# Autodesk Inventor assembly: Battery holder assembly
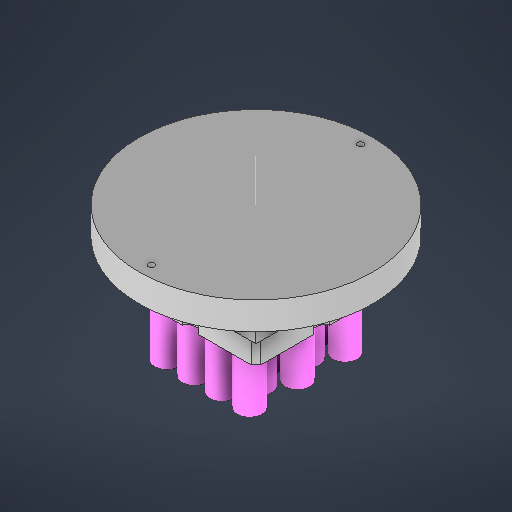
[picture p0: Inventor's stored thumbnail of the model, 512x512]
Saved by Autodesk Inventor 2025 (Build 290162000, 162)
## iProperties
Created: 2025-08-08
Part Number: Battery holder assembly
Document SubType Name: Assembly
Designer: mayhe
Author: mayhe
## Documents named in this file (4)
- C:\Users\mayhe\OneDrive\Documents\GitHub\In-situ-monitoring-of-powder-bed-fusion-additive-manufacturing\accessories\Battery Holder\Battery holder assembly.iam
- C:\Users\mayhe\OneDrive\Documents\GitHub\In-situ-monitoring-of-powder-bed-fusion-additive-manufacturing\accessories\threaded_build-plate\substrate plate With Lots of holes.ipt
- C:\Users\mayhe\OneDrive\Documents\GitHub\In-situ-monitoring-of-powder-bed-fusion-additive-manufacturing\accessories\Battery Holder\Battery Holder.ipt
- C:\Users\mayhe\OneDrive\Documents\GitHub\In-situ-monitoring-of-powder-bed-fusion-additive-manufacturing\accessories\Battery Holder\18650(PINK).ipt
## Components (20 placed, 3 different names)
1. substrate plate With Lots of holes:1 — Rotational:3, Mate:1
2. Battery Holder:1 — Rotational:2, Rotational:3, Mate:1, Rotational:4, Rotational:5, Rotational:6, Rotational:7, Rotational:8, Rotational:9, Rotational:10, Rotational:11, Rotational:12, Rigid:1, Rotational:13, Rigid:2, Rotational:14, Rotational:15, Rigid:3, Rotational:16, Rotational:17
3. 18650(PINK):1 — Rotational:2
4. 18650(PINK):2 — Rigid:2
5. 18650(PINK):3 — Rigid:3
6. 18650(PINK):4 — Rotational:15
7. 18650(PINK):5 — Rotational:14
8. 18650(PINK):6 — Rotational:7
9. 18650(PINK):7 — Rotational:9
10. 18650(PINK):8 — Rotational:10
11. 18650(PINK):9 — Rotational:11
12. 18650(PINK):10 — Rotational:12
13. 18650(PINK):11 — Rigid:1
14. 18650(PINK):12 — Rotational:13
15. 18650(PINK):13 — Rotational:8
16. 18650(PINK):14 — Rotational:16
17. 18650(PINK):15 — Rotational:6
18. 18650(PINK):16 — Rotational:5
19. 18650(PINK):17 — Rotational:4
20. 18650(PINK):18 — Rotational:17
## Relationships (20: RevoluteJoint 16, WeldJoint 3, Mate 1)
- Rotational:2 [RevoluteJoint]: Battery Holder:1 ↔ 18650(PINK):1
- Rotational:3 [RevoluteJoint]: substrate plate With Lots of holes:1 ↔ Battery Holder:1
- Mate:1: substrate plate With Lots of holes:1 ↔ Battery Holder:1
- Rotational:4 [RevoluteJoint]: Battery Holder:1 ↔ 18650(PINK):17
- Rotational:5 [RevoluteJoint]: Battery Holder:1 ↔ 18650(PINK):16
- Rotational:6 [RevoluteJoint]: Battery Holder:1 ↔ 18650(PINK):15
- Rotational:7 [RevoluteJoint]: Battery Holder:1 ↔ 18650(PINK):6
- Rotational:8 [RevoluteJoint]: Battery Holder:1 ↔ 18650(PINK):13
- Rotational:9 [RevoluteJoint]: Battery Holder:1 ↔ 18650(PINK):7
- Rotational:10 [RevoluteJoint]: Battery Holder:1 ↔ 18650(PINK):8
- Rotational:11 [RevoluteJoint]: Battery Holder:1 ↔ 18650(PINK):9
- Rotational:12 [RevoluteJoint]: Battery Holder:1 ↔ 18650(PINK):10
- Rigid:1 [WeldJoint]: Battery Holder:1 ↔ 18650(PINK):11
- Rotational:13 [RevoluteJoint]: Battery Holder:1 ↔ 18650(PINK):12
- Rigid:2 [WeldJoint]: Battery Holder:1 ↔ 18650(PINK):2
- Rotational:14 [RevoluteJoint]: Battery Holder:1 ↔ 18650(PINK):5
- Rotational:15 [RevoluteJoint]: Battery Holder:1 ↔ 18650(PINK):4
- Rigid:3 [WeldJoint]: Battery Holder:1 ↔ 18650(PINK):3
- Rotational:16 [RevoluteJoint]: Battery Holder:1 ↔ 18650(PINK):14
- Rotational:17 [RevoluteJoint]: Battery Holder:1 ↔ 18650(PINK):18
